# Autodesk Inventor assembly: testRoboRescue_Chassis_Frame
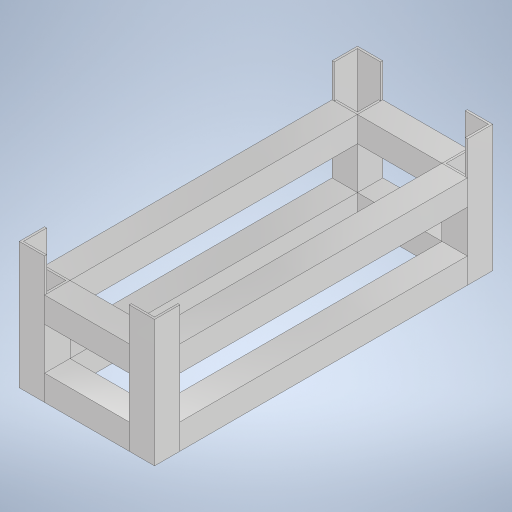
[picture p0: Inventor's stored thumbnail of the model, 512x512]
Saved by Autodesk Inventor 2023 (Build 270158000, 158)
## iProperties
Created: 2022-03-14
Part Number: testRoboRescue_Chassis_Frame
Document SubType Name: Assembly
Designer: Nebil Oumer
Author: Nebil Oumer
## Documents named in this file (4)
- C:\Users\seene\Desktop\Stony Brook\SBRT\testRoboRescue\Chassis\Frame\testRoboRescue_Chassis_Frame.iam
- C:\Users\seene\Desktop\Stony Brook\SBRT\testRoboRescue\Chassis\Frame\testRoboRescue_Chassis_Frame_heightBar.ipt
- C:\Users\seene\Desktop\Stony Brook\SBRT\testRoboRescue\Chassis\Frame\testRoboRescue_Chassis_Frame_widthBar.ipt
- C:\Users\seene\Desktop\Stony Brook\SBRT\testRoboRescue\Chassis\Frame\testRoboRescue_Chassis_Frame_lengthBar.ipt
## Components (12 placed, 3 different names)
1. testRoboRescue_Chassis_Frame_heightBar:1 — Flush:1, Flush:2, Mate:1, Flush:3, Mate:2, Flush:4, Flush:9, Mate:5, Flush:10, Mate:9, Flush:17, Flush:18, Symmetry:2
2. testRoboRescue_Chassis_Frame_heightBar:2 — Mate:6, Flush:11, Flush:12, Mate:10, Mate:11, Symmetry:1
3. testRoboRescue_Chassis_Frame_heightBar:3 — Mate:3, Flush:5, Flush:6, Flush:7, Flush:8, Mate:4, Mate:8, Symmetry:2
4. testRoboRescue_Chassis_Frame_heightBar:4 — Mate:7, Flush:13, Flush:14, Flush:15, Flush:16, Flush:19, Flush:20, Flush:21, Flush:22, Symmetry:1
5. testRoboRescue_Chassis_Frame_widthBar:1 — Mate:9, Flush:17, Flush:18
6. testRoboRescue_Chassis_Frame_widthBar:2 — Flush:15, Flush:16, Mate:8
7. testRoboRescue_Chassis_Frame_widthBar:3 — Flush:1, Flush:2, Mate:1, Mate:6, Flush:11, Flush:12
8. testRoboRescue_Chassis_Frame_widthBar:4 — Flush:7, Flush:8, Mate:4, Mate:7, Flush:13, Flush:14
9. testRoboRescue_Chassis_Frame_lengthBar:1 — Flush:9, Mate:5, Flush:10
10. testRoboRescue_Chassis_Frame_lengthBar:2 — Flush:21, Flush:22, Mate:11
11. testRoboRescue_Chassis_Frame_lengthBar:3 — Flush:3, Mate:2, Flush:4, Mate:3, Flush:5, Flush:6
12. testRoboRescue_Chassis_Frame_lengthBar:4 — Flush:19, Mate:10, Flush:20
## Relationships (36: Flush 22, Mate 11, Symmetry 3)
- Flush:1: testRoboRescue_Chassis_Frame_heightBar:1 ↔ testRoboRescue_Chassis_Frame_widthBar:3
- Flush:2: testRoboRescue_Chassis_Frame_heightBar:1 ↔ testRoboRescue_Chassis_Frame_widthBar:3
- Mate:1: testRoboRescue_Chassis_Frame_heightBar:1 ↔ testRoboRescue_Chassis_Frame_widthBar:3
- Flush:3: testRoboRescue_Chassis_Frame_heightBar:1 ↔ testRoboRescue_Chassis_Frame_lengthBar:3
- Mate:2: testRoboRescue_Chassis_Frame_heightBar:1 ↔ testRoboRescue_Chassis_Frame_lengthBar:3
- Flush:4: testRoboRescue_Chassis_Frame_heightBar:1 ↔ testRoboRescue_Chassis_Frame_lengthBar:3
- Mate:3: testRoboRescue_Chassis_Frame_heightBar:3 ↔ testRoboRescue_Chassis_Frame_lengthBar:3
- Flush:5: testRoboRescue_Chassis_Frame_heightBar:3 ↔ testRoboRescue_Chassis_Frame_lengthBar:3
- Flush:6: testRoboRescue_Chassis_Frame_heightBar:3 ↔ testRoboRescue_Chassis_Frame_lengthBar:3
- Flush:7: testRoboRescue_Chassis_Frame_heightBar:3 ↔ testRoboRescue_Chassis_Frame_widthBar:4
- Flush:8: testRoboRescue_Chassis_Frame_heightBar:3 ↔ testRoboRescue_Chassis_Frame_widthBar:4
- Mate:4: testRoboRescue_Chassis_Frame_heightBar:3 ↔ testRoboRescue_Chassis_Frame_widthBar:4
- Flush:9: testRoboRescue_Chassis_Frame_heightBar:1 ↔ testRoboRescue_Chassis_Frame_lengthBar:1
- Mate:5: testRoboRescue_Chassis_Frame_heightBar:1 ↔ testRoboRescue_Chassis_Frame_lengthBar:1
- Flush:10: testRoboRescue_Chassis_Frame_heightBar:1 ↔ testRoboRescue_Chassis_Frame_lengthBar:1
- Mate:6: testRoboRescue_Chassis_Frame_heightBar:2 ↔ testRoboRescue_Chassis_Frame_widthBar:3
- Flush:11: testRoboRescue_Chassis_Frame_heightBar:2 ↔ testRoboRescue_Chassis_Frame_widthBar:3
- Flush:12: testRoboRescue_Chassis_Frame_heightBar:2 ↔ testRoboRescue_Chassis_Frame_widthBar:3
- Mate:7: testRoboRescue_Chassis_Frame_heightBar:4 ↔ testRoboRescue_Chassis_Frame_widthBar:4
- Flush:13: testRoboRescue_Chassis_Frame_heightBar:4 ↔ testRoboRescue_Chassis_Frame_widthBar:4
- Flush:14: testRoboRescue_Chassis_Frame_heightBar:4 ↔ testRoboRescue_Chassis_Frame_widthBar:4
- Flush:15: testRoboRescue_Chassis_Frame_heightBar:4 ↔ testRoboRescue_Chassis_Frame_widthBar:2
- Flush:16: testRoboRescue_Chassis_Frame_heightBar:4 ↔ testRoboRescue_Chassis_Frame_widthBar:2
- Mate:8: testRoboRescue_Chassis_Frame_heightBar:3 ↔ testRoboRescue_Chassis_Frame_widthBar:2
- Mate:9: testRoboRescue_Chassis_Frame_heightBar:1 ↔ testRoboRescue_Chassis_Frame_widthBar:1
- Flush:17: testRoboRescue_Chassis_Frame_heightBar:1 ↔ testRoboRescue_Chassis_Frame_widthBar:1
- Flush:18: testRoboRescue_Chassis_Frame_heightBar:1 ↔ testRoboRescue_Chassis_Frame_widthBar:1
- Flush:19: testRoboRescue_Chassis_Frame_heightBar:4 ↔ testRoboRescue_Chassis_Frame_lengthBar:4
- Mate:10: testRoboRescue_Chassis_Frame_heightBar:2 ↔ testRoboRescue_Chassis_Frame_lengthBar:4
- Flush:20: testRoboRescue_Chassis_Frame_heightBar:4 ↔ testRoboRescue_Chassis_Frame_lengthBar:4
- Flush:21: testRoboRescue_Chassis_Frame_heightBar:4 ↔ testRoboRescue_Chassis_Frame_lengthBar:2
- Flush:22: testRoboRescue_Chassis_Frame_heightBar:4 ↔ testRoboRescue_Chassis_Frame_lengthBar:2
- Mate:11: testRoboRescue_Chassis_Frame_heightBar:2 ↔ testRoboRescue_Chassis_Frame_lengthBar:2
- Symmetry:1: testRoboRescue_Chassis_Frame_heightBar:2 ↔ testRoboRescue_Chassis_Frame_heightBar:4
- Symmetry:2: testRoboRescue_Chassis_Frame_heightBar:1 ↔ testRoboRescue_Chassis_Frame_heightBar:3
- Symmetry:3
